# Autodesk Inventor assembly: mirror
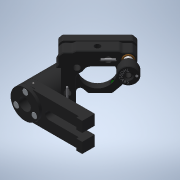
[picture p0: Inventor's stored thumbnail of the model, 180x180]
Saved by Autodesk Inventor 2020 (Build 240168000, 168)
## iProperties
Created: 2016-10-07
Part Number: mirror
Document SubType Name: Assembly
Designer: i7
Author: i7
## Documents named in this file (4)
- C:\LAFriOC\diseños\sistema de vacío\Óptica para la MOT\Colimadores para MOT\mirror.iam
- C:\LAFriOC\diseños\sistema de vacío\Óptica para la MOT\Colimadores para MOT\MA45-50_M-Solidworks.ipt
- C:\LAFriOC\diseños\sistema de vacío\Óptica para la MOT\Colimadores para MOT\KM100-Solidworks.ipt
- C:\LAFriOC\diseños\sistema de vacío\Óptica para la MOT\Colimadores para MOT\UPHA-Solidworks.ipt
## Components (3 placed, 3 different names)
1. MA45-50_M-Solidworks:1 — De rotación:1, De rotación:2
2. KM100-Solidworks:1 — De rotación:1
3. UPHA-Solidworks:1 — De rotación:2
## Relationships (2: RevoluteJoint 2)
- De rotación:1 [RevoluteJoint]: MA45-50_M-Solidworks:1 ↔ KM100-Solidworks:1
- De rotación:2 [RevoluteJoint]: MA45-50_M-Solidworks:1 ↔ UPHA-Solidworks:1
